# Autodesk Inventor assembly: 足全体
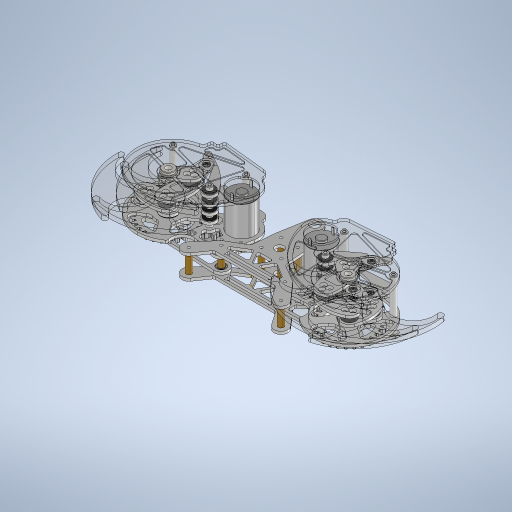
[picture p0: Inventor's stored thumbnail of the model, 512x512]
Saved by Autodesk Inventor 2023 (Build 270158000, 158)
## iProperties
Created: 2022-01-30
Part Number: 足全体
Document SubType Name: Assembly
Designer: acps
Author: acps
## Documents named in this file (6)
- C:\Users\acps\Documents\srdc\srdc_ksh\脚\足全体.iam
- C:\Users\acps\Documents\srdc\srdc_ksh\脚\足ユニット.iam
- C:\Users\acps\Documents\srdc\srdc_ksh\脚\中間ユニット内.ipt
- C:\Users\acps\Documents\srdc\srdc_ksh\スペーサ\l23.ipt
- C:\Users\acps\Documents\srdc\srdc_ksh\脚\足ユニット_MIR.iam
- C:\Users\acps\Documents\srdc\srdc_ksh\脚\中間ユニット内_MIR.ipt
## Components (12 placed, 5 different names)
1. 足ユニット:1 [sub-assembly] — Mate:1, Insert:11
2. l23:1 — Insert:7, Insert:10
3. l23:2 — Insert:6
4. l23:3 — Insert:2
5. l23:4 — Insert:3
6. 足ユニット_MIR:1 [sub-assembly] — Mate:2, Insert:12
7. l23:5 — Insert:8
8. l23:6 — Insert:5, Insert:9
9. l23:7 — Insert:4
10. l23:8 — Insert:1
11. 中間ユニット内_MIR:1 — Insert:9, Insert:10, Mate:1, Insert:11, Mate:2, Insert:12
12. 中間ユニット内:1 — Insert:1, Insert:2, Insert:3, Insert:4, Insert:5, Insert:6, Insert:7, Insert:8
## Relationships (14: Insert 12, Mate 2)
- Insert:1: l23:8 ↔ 中間ユニット内:1
- Insert:2: l23:3 ↔ 中間ユニット内:1
- Insert:3: l23:4 ↔ 中間ユニット内:1
- Insert:4: l23:7 ↔ 中間ユニット内:1
- Insert:5: l23:6 ↔ 中間ユニット内:1
- Insert:6: l23:2 ↔ 中間ユニット内:1
- Insert:7: l23:1 ↔ 中間ユニット内:1
- Insert:8: l23:5 ↔ 中間ユニット内:1
- Insert:9: l23:6 ↔ 中間ユニット内_MIR:1
- Insert:10: l23:1 ↔ 中間ユニット内_MIR:1
- Mate:1: 足ユニット:1 ↔ 中間ユニット内_MIR:1
- Insert:11: 足ユニット:1 ↔ 中間ユニット内_MIR:1
- Mate:2: 足ユニット_MIR:1 ↔ 中間ユニット内_MIR:1
- Insert:12: 足ユニット_MIR:1 ↔ 中間ユニット内_MIR:1
